# Autodesk Inventor assembly: FullRadiusPole_x2_AJB
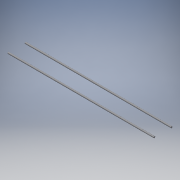
[picture p0: Inventor's stored thumbnail of the model, 180x180]
Saved by Autodesk Inventor 2018 (Build 220112000, 112)
## iProperties
Created: 2018-02-16
Part Number: FullRadiusPole_x2_AJB
Document SubType Name: Assembly
Designer: Alec temporary
Author: Alec temporary
## Documents named in this file (2)
- M:\TPS\9th Grade\CADD 2017-2018\Current\Ferris Wheel Group Project\Group Project Week 3\FullRadiusPole_x2_AJB.iam
- M:\TPS\9th Grade\CADD 2017-2018\Current\Ferris Wheel Group Project\Group Project Week 3\FullRadiusPoleAJB.iam
## Components (2 placed, 1 different names)
1. FullRadiusPoleAJB:1 [sub-assembly] — Flush:1, Mate:1, Flush:2
2. FullRadiusPoleAJB:2 [sub-assembly] — Flush:1, Mate:1, Flush:2
## Relationships (3: Flush 2, Mate 1)
- Flush:1: FullRadiusPoleAJB:1 ↔ FullRadiusPoleAJB:2
- Mate:1: FullRadiusPoleAJB:1 ↔ FullRadiusPoleAJB:2
- Flush:2 (-2692.4 mm): FullRadiusPoleAJB:1 ↔ FullRadiusPoleAJB:2
